# Autodesk Inventor assembly: 新款V5四方轴套
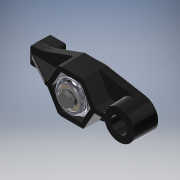
[picture p0: Inventor's stored thumbnail of the model, 180x180]
Saved by Autodesk Inventor 2019.4 (Build 234330000, 330)
## iProperties
Created: 2019-03-29
Part Number: 新款V5四方轴套
Material: 常规
Document SubType Name: Assembly
Designer: aresp
Mass: 3.74505 g
Surface Area: 17.7562 cm^2
Volume: 1.33109 cm^3
Density: 2.81353 g/cm^3
Author: aresp
## Documents named in this file (4)
- C:\towerTakeOverCad\ncrCadLib\新款V5四方轴套.iam
- C:\towerTakeOverCad\ncrCadLib\垫片轴套大白等\1-Post_Hex_Nut_Retainer_w_Bearing_Flat_276-6481.ipt
- C:\towerTakeOverCad\ncrCadLib\螺丝螺帽\Nut 8-32 Nylock.ipt
- C:\towerTakeOverCad\ncrCadLib\螺丝螺帽\Screw 8-32 x 0.375'' - Black.ipt
## Components (3 placed, 3 different names)
1. 1-Post_Hex_Nut_Retainer_w_Bearing_Flat_276-6481:1 — 配合:1, 配合:2, 配合:4
2. Nut 8-32 Nylock:1 — 配合:3, 配合:4
3. Screw 8-32 x 0.375'' - Black:1 — 配合:1, 配合:2, 配合:3
## Relationships (4: Mate 4)
- 配合:1 [Mate] (1.575 mm): 1-Post_Hex_Nut_Retainer_w_Bearing_Flat_276-6481:1 ↔ Screw 8-32 x 0.375'' - Black:1
- 配合:2 [Mate]: 1-Post_Hex_Nut_Retainer_w_Bearing_Flat_276-6481:1 ↔ Screw 8-32 x 0.375'' - Black:1
- 配合:3 [Mate]: Nut 8-32 Nylock:1 ↔ Screw 8-32 x 0.375'' - Black:1
- 配合:4 [Mate]: 1-Post_Hex_Nut_Retainer_w_Bearing_Flat_276-6481:1 ↔ Nut 8-32 Nylock:1
